# Autodesk Inventor assembly: SmartEgg
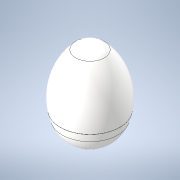
[picture p0: Inventor's stored thumbnail of the model, 180x180]
Saved by Autodesk Inventor 2020 (Build 240168000, 168)
## iProperties
Created: 2019-11-26
Part Number: SmartEgg
Document SubType Name: Assembly
Designer: Andrew
Author: Andrew
## Documents named in this file (6)
- C:\Users\Andrew\Documents\projects\SmartEgg\CAD\SmartEgg.iam
- C:\Users\Andrew\Documents\projects\SmartEgg\CAD\ESP32 Feather.ipt
- C:\Users\Andrew\Documents\projects\SmartEgg\CAD\SmartEgg Housing Main.ipt
- C:\Users\Andrew\Documents\projects\SmartEgg\CAD\SmartEgg Housing Cap.ipt
- C:\Users\Andrew\Documents\projects\SmartEgg\CAD\SmartEgg Shell Top.ipt
- C:\Users\Andrew\Documents\projects\SmartEgg\CAD\SmartEgg Shell.ipt
## Components (5 placed, 5 different names)
1. ESP32 Feather:1 — Flush:1, Flush:2, Flush:3
2. SmartEgg Housing Main:1 — Flush:4, Flush:5, Flush:6
3. SmartEgg Housing Cap:1 — Flush:7, Flush:8, Flush:9
4. SmartEgg Shell Top:1 — Flush:13, Flush:14
5. SmartEgg Shell:1 — Flush:10, Flush:11, Flush:12
## Relationships (14: Flush 14)
- Flush:1: ESP32 Feather:1
- Flush:2: ESP32 Feather:1
- Flush:3: ESP32 Feather:1
- Flush:4: SmartEgg Housing Main:1
- Flush:5: SmartEgg Housing Main:1
- Flush:6: SmartEgg Housing Main:1
- Flush:7: SmartEgg Housing Cap:1
- Flush:8: SmartEgg Housing Cap:1
- Flush:9: SmartEgg Housing Cap:1
- Flush:10: SmartEgg Shell:1
- Flush:11: SmartEgg Shell:1
- Flush:12: SmartEgg Shell:1
- Flush:13: SmartEgg Shell Top:1
- Flush:14: SmartEgg Shell Top:1
